# Autodesk Inventor assembly: Lower Frame 4x4
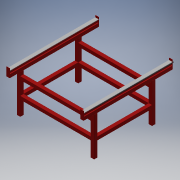
[picture p0: Inventor's stored thumbnail of the model, 180x180]
Saved by Autodesk Inventor 2018.2 (Build 222227000, 227)
## iProperties
Created: 2017-12-10
Part Number: Lower Frame 4x4
Document SubType Name: Assembly
Designer: torba
Author: torba
## Documents named in this file (13)
- C:\Users\torba\OneDrive\Documents\Inventor\Plasma 5x10\Lower Frame 4x4.iam
- C:\Users\torba\OneDrive\Documents\Inventor\Plasma 5x10\3 X 3 X .125 WALL SQ TUBE.ipt
- C:\Users\torba\OneDrive\Documents\Inventor\Plasma 5x10\3 X 3 X .125 WALL SQ TUBE\3 X 3 X .125 WALL SQ TUBE-13.ipt
- C:\Users\torba\OneDrive\Documents\Inventor\Plasma 5x10\0.25 X 3 HOT ROLLED STEEL.ipt
- C:\Users\torba\OneDrive\Documents\Inventor\Plasma 5x10\3-8 x 3 cold rolled steel.ipt
- C:\Users\torba\OneDrive\Documents\Inventor\Plasma 5x10\3 X 3 X .125 WALL SQ TUBE\3 X 3 X .125 WALL SQ TUBE-09.ipt
- C:\Users\torba\OneDrive\Documents\Inventor\Plasma 5x10\3 X 3 X .125 WALL SQ TUBE\3 X 3 X .125 WALL SQ TUBE-04.ipt
- C:\Users\torba\OneDrive\Documents\Inventor\Plasma 5x10\1.5 X 2.5 X .125 WALL SQ TUBE.ipt
- C:\Users\torba\OneDrive\Documents\Inventor\Plasma 5x10\RSHC10XX00 Rack (Simplified).ipt
- C:\Users\torba\OneDrive\Documents\Inventor\Plasma 5x10\3 X 3 X .125 WALL SQ TUBE\3 X 3 X .125 WALL SQ TUBE-78.ipt
- C:\Users\torba\OneDrive\Documents\Inventor\Plasma 5x10\1.5 X 2.5 X .125 WALL SQ TUBE\1.5 X 2.5 X .125 WALL SQ TUBE-78.ipt
- C:\Users\torba\OneDrive\Documents\Inventor\Plasma 5x10\3-8 x 3 cold rolled steel\3-8 x 3 cold rolled steel-78.ipt
- C:\Users\torba\OneDrive\Documents\Inventor\Plasma 5x10\RSHC10XX00 Rack (Simplified)\RSHC10XX00 Rack (Simplified)-72.ipt
## Components (22 placed, 8 different names)
1. 1.5 X 2.5 X .125 WALL SQ TUBE-78:4 — Mate:17, Mate:18, Mate:19, Flush:37
2. 1.5 X 2.5 X .125 WALL SQ TUBE-78:3 — Mate:16, Mate:20, Mate:21, Flush:36
3. 3 X 3 X .125 WALL SQ TUBE-78:1 — Flush:1, Flush:2, Mate:8, Flush:20, Mate:9, Mate:11, Mate:12, Flush:24, Flush:27, Flush:28, Flush:29, Flush:32, Mate:21
4. 3 X 3 X .125 WALL SQ TUBE-78:2 — Flush:8, Flush:9, Mate:4, Mate:5, Flush:20, Flush:24, Flush:25, Flush:26, Flush:30, Flush:31, Mate:19, Flush:37
5. 3 X 3 X .125 WALL SQ TUBE-04:4 — Flush:5, Flush:6, Flush:13, Mate:3, Flush:22, Mate:15
6. 3 X 3 X .125 WALL SQ TUBE-09:5 — Flush:3, Flush:18, Flush:19, Mate:7, Mate:10
7. 3 X 3 X .125 WALL SQ TUBE-09:6 — Flush:10, Flush:11, Flush:12, Mate:2
8. 3 X 3 X .125 WALL SQ TUBE-04:7 — Flush:4, Flush:7, Flush:12, Flush:19
9. 3 X 3 X .125 WALL SQ TUBE-04:9 — Flush:4, Flush:6, Flush:13, Flush:21, Flush:23
10. 3 X 3 X .125 WALL SQ TUBE-04:10 — Flush:5, Flush:7, Flush:11, Mate:1, Flush:16, Mate:6, Flush:18, Flush:35, Mate:15
11. 3 X 3 X .125 WALL SQ TUBE-13:11 — Flush:2, Flush:3, Flush:17, Mate:7, Mate:8, Flush:23
12. 3 X 3 X .125 WALL SQ TUBE-13:12 — Flush:1, Flush:16, Mate:6, Mate:9, Mate:10, Flush:35
13. 3 X 3 X .125 WALL SQ TUBE-13:13 — Flush:9, Flush:10, Mate:5, Flush:21
14. 3 X 3 X .125 WALL SQ TUBE-13:14 — Flush:8, Mate:1, Mate:2, Mate:3, Mate:4, Flush:22
15. 0.25 X 3 HOT ROLLED STEEL:1 — Flush:14, Flush:25, Flush:26, Mate:17
16. 0.25 X 3 HOT ROLLED STEEL:2 — Flush:14, Mate:11, Flush:27, Flush:28, Mate:16, Mate:22
17. 0.25 X 3 HOT ROLLED STEEL:3 — Flush:15, Flush:17, Mate:12, Flush:29, Flush:32, Mate:13, Flush:34, Flush:36
18. 0.25 X 3 HOT ROLLED STEEL:4 — Flush:15, Flush:30, Flush:31, Mate:14, Flush:33
19. 3-8 x 3 cold rolled steel-78:1 — Mate:13, Flush:34, Mate:20, Mate:23, Flush:40
20. 3-8 x 3 cold rolled steel-78:2 — Mate:14, Flush:33, Mate:18, Flush:41
21. RSHC10XX00 Rack (Simplified)-72:1 — Flush:39, Flush:40, Flush:42
22. RSHC10XX00 Rack (Simplified)-72:2 — Flush:39, Mate:22, Mate:23, Flush:41, Flush:42
## Relationships (64: Flush 41, Mate 23)
- Flush:1: 3 X 3 X .125 WALL SQ TUBE-78:1 ↔ 3 X 3 X .125 WALL SQ TUBE-13:12
- Flush:2: 3 X 3 X .125 WALL SQ TUBE-78:1 ↔ 3 X 3 X .125 WALL SQ TUBE-13:11
- Flush:3: 3 X 3 X .125 WALL SQ TUBE-09:5 ↔ 3 X 3 X .125 WALL SQ TUBE-13:11
- Flush:4: 3 X 3 X .125 WALL SQ TUBE-04:7 ↔ 3 X 3 X .125 WALL SQ TUBE-04:9
- Flush:5: 3 X 3 X .125 WALL SQ TUBE-04:4 ↔ 3 X 3 X .125 WALL SQ TUBE-04:10
- Flush:6: 3 X 3 X .125 WALL SQ TUBE-04:4 ↔ 3 X 3 X .125 WALL SQ TUBE-04:9
- Flush:7: 3 X 3 X .125 WALL SQ TUBE-04:7 ↔ 3 X 3 X .125 WALL SQ TUBE-04:10
- Flush:8: 3 X 3 X .125 WALL SQ TUBE-78:2 ↔ 3 X 3 X .125 WALL SQ TUBE-13:14
- Flush:9: 3 X 3 X .125 WALL SQ TUBE-78:2 ↔ 3 X 3 X .125 WALL SQ TUBE-13:13
- Flush:10: 3 X 3 X .125 WALL SQ TUBE-09:6 ↔ 3 X 3 X .125 WALL SQ TUBE-13:13
- Flush:11: 3 X 3 X .125 WALL SQ TUBE-09:6 ↔ 3 X 3 X .125 WALL SQ TUBE-04:10
- Flush:12: 3 X 3 X .125 WALL SQ TUBE-09:6 ↔ 3 X 3 X .125 WALL SQ TUBE-04:7
- Flush:13: 3 X 3 X .125 WALL SQ TUBE-04:4 ↔ 3 X 3 X .125 WALL SQ TUBE-04:9
- Flush:14: 0.25 X 3 HOT ROLLED STEEL:1 ↔ 0.25 X 3 HOT ROLLED STEEL:2
- Flush:15: 0.25 X 3 HOT ROLLED STEEL:3 ↔ 0.25 X 3 HOT ROLLED STEEL:4
- Mate:1: 3 X 3 X .125 WALL SQ TUBE-04:10 ↔ 3 X 3 X .125 WALL SQ TUBE-13:14
- Mate:2: 3 X 3 X .125 WALL SQ TUBE-09:6 ↔ 3 X 3 X .125 WALL SQ TUBE-13:14
- Mate:3: 3 X 3 X .125 WALL SQ TUBE-04:4 ↔ 3 X 3 X .125 WALL SQ TUBE-13:14
- Mate:4: 3 X 3 X .125 WALL SQ TUBE-78:2 ↔ 3 X 3 X .125 WALL SQ TUBE-13:14
- Mate:5: 3 X 3 X .125 WALL SQ TUBE-78:2 ↔ 3 X 3 X .125 WALL SQ TUBE-13:13
- Flush:16: 3 X 3 X .125 WALL SQ TUBE-04:10 ↔ 3 X 3 X .125 WALL SQ TUBE-13:12
- Mate:6: 3 X 3 X .125 WALL SQ TUBE-04:10 ↔ 3 X 3 X .125 WALL SQ TUBE-13:12
- Flush:17 (-387.35 mm): 3 X 3 X .125 WALL SQ TUBE-13:11 ↔ 0.25 X 3 HOT ROLLED STEEL:3
- Flush:18: 3 X 3 X .125 WALL SQ TUBE-09:5 ↔ 3 X 3 X .125 WALL SQ TUBE-04:10
- Flush:19: 3 X 3 X .125 WALL SQ TUBE-09:5 ↔ 3 X 3 X .125 WALL SQ TUBE-04:7
- Mate:7: 3 X 3 X .125 WALL SQ TUBE-09:5 ↔ 3 X 3 X .125 WALL SQ TUBE-13:11
- Mate:8: 3 X 3 X .125 WALL SQ TUBE-78:1 ↔ 3 X 3 X .125 WALL SQ TUBE-13:11
- Flush:20: 3 X 3 X .125 WALL SQ TUBE-78:1 ↔ 3 X 3 X .125 WALL SQ TUBE-78:2
- Mate:9: 3 X 3 X .125 WALL SQ TUBE-78:1 ↔ 3 X 3 X .125 WALL SQ TUBE-13:12
- Flush:21: 3 X 3 X .125 WALL SQ TUBE-04:9 ↔ 3 X 3 X .125 WALL SQ TUBE-13:13
- Flush:22: 3 X 3 X .125 WALL SQ TUBE-04:4 ↔ 3 X 3 X .125 WALL SQ TUBE-13:14
- Flush:23: 3 X 3 X .125 WALL SQ TUBE-04:9 ↔ 3 X 3 X .125 WALL SQ TUBE-13:11
- Mate:10: 3 X 3 X .125 WALL SQ TUBE-09:5 ↔ 3 X 3 X .125 WALL SQ TUBE-13:12
- Mate:11: 3 X 3 X .125 WALL SQ TUBE-78:1 ↔ 0.25 X 3 HOT ROLLED STEEL:2
- Mate:12: 3 X 3 X .125 WALL SQ TUBE-78:1 ↔ 0.25 X 3 HOT ROLLED STEEL:3
- Flush:24: 3 X 3 X .125 WALL SQ TUBE-78:1 ↔ 3 X 3 X .125 WALL SQ TUBE-78:2
- Flush:25: 3 X 3 X .125 WALL SQ TUBE-78:2 ↔ 0.25 X 3 HOT ROLLED STEEL:1
- Flush:26: 3 X 3 X .125 WALL SQ TUBE-78:2 ↔ 0.25 X 3 HOT ROLLED STEEL:1
- Flush:27: 3 X 3 X .125 WALL SQ TUBE-78:1 ↔ 0.25 X 3 HOT ROLLED STEEL:2
- Flush:28: 3 X 3 X .125 WALL SQ TUBE-78:1 ↔ 0.25 X 3 HOT ROLLED STEEL:2
- Flush:29: 3 X 3 X .125 WALL SQ TUBE-78:1 ↔ 0.25 X 3 HOT ROLLED STEEL:3
- Flush:30: 3 X 3 X .125 WALL SQ TUBE-78:2 ↔ 0.25 X 3 HOT ROLLED STEEL:4
- Flush:31: 3 X 3 X .125 WALL SQ TUBE-78:2 ↔ 0.25 X 3 HOT ROLLED STEEL:4
- Flush:32: 3 X 3 X .125 WALL SQ TUBE-78:1 ↔ 0.25 X 3 HOT ROLLED STEEL:3
- Mate:13: 0.25 X 3 HOT ROLLED STEEL:3 ↔ 3-8 x 3 cold rolled steel-78:1
- Mate:14: 0.25 X 3 HOT ROLLED STEEL:4 ↔ 3-8 x 3 cold rolled steel-78:2
- Flush:33: 0.25 X 3 HOT ROLLED STEEL:4 ↔ 3-8 x 3 cold rolled steel-78:2
- Flush:34: 0.25 X 3 HOT ROLLED STEEL:3 ↔ 3-8 x 3 cold rolled steel-78:1
- Flush:35 (330.2 mm): 3 X 3 X .125 WALL SQ TUBE-04:10 ↔ 3 X 3 X .125 WALL SQ TUBE-13:12
- Mate:15 (304.8 mm): 3 X 3 X .125 WALL SQ TUBE-04:4 ↔ 3 X 3 X .125 WALL SQ TUBE-04:10
- Mate:16: 1.5 X 2.5 X .125 WALL SQ TUBE-78:3 ↔ 0.25 X 3 HOT ROLLED STEEL:2
- Mate:17: 1.5 X 2.5 X .125 WALL SQ TUBE-78:4 ↔ 0.25 X 3 HOT ROLLED STEEL:1
- Mate:18: 1.5 X 2.5 X .125 WALL SQ TUBE-78:4 ↔ 3-8 x 3 cold rolled steel-78:2
- Mate:19: 1.5 X 2.5 X .125 WALL SQ TUBE-78:4 ↔ 3 X 3 X .125 WALL SQ TUBE-78:2
- Mate:20: 1.5 X 2.5 X .125 WALL SQ TUBE-78:3 ↔ 3-8 x 3 cold rolled steel-78:1
- Mate:21: 1.5 X 2.5 X .125 WALL SQ TUBE-78:3 ↔ 3 X 3 X .125 WALL SQ TUBE-78:1
- Flush:36 (19.05 mm): 1.5 X 2.5 X .125 WALL SQ TUBE-78:3 ↔ 0.25 X 3 HOT ROLLED STEEL:3
- Flush:37 (19.05 mm): 1.5 X 2.5 X .125 WALL SQ TUBE-78:4 ↔ 3 X 3 X .125 WALL SQ TUBE-78:2
- Flush:39: RSHC10XX00 Rack (Simplified)-72:1 ↔ RSHC10XX00 Rack (Simplified)-72:2
- Mate:22 (177.8 mm): 0.25 X 3 HOT ROLLED STEEL:2 ↔ RSHC10XX00 Rack (Simplified)-72:2
- Mate:23: 3-8 x 3 cold rolled steel-78:1 ↔ RSHC10XX00 Rack (Simplified)-72:2
- Flush:40: 3-8 x 3 cold rolled steel-78:1 ↔ RSHC10XX00 Rack (Simplified)-72:1
- Flush:41: 3-8 x 3 cold rolled steel-78:2 ↔ RSHC10XX00 Rack (Simplified)-72:2
- Flush:42: RSHC10XX00 Rack (Simplified)-72:1 ↔ RSHC10XX00 Rack (Simplified)-72:2
